# Autodesk Inventor assembly: Solarbotics-GM2_Assem
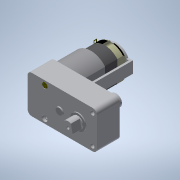
[picture p0: Inventor's stored thumbnail of the model, 180x180]
Saved by Autodesk Inventor 2020.1 (Build 241239000, 239)
## iProperties
Created: 2013-04-23
Part Number: Solarbotics-GM2_Assem
Document SubType Name: Assembly
Designer: justin
## Documents named in this file (7)
- C:\Users\amirs\OneDrive - UC San Diego\college\freshman year\MAE 3\robot\gm 2\Solarbotics-GM2_Assem.iam
- C:\Users\amirs\OneDrive - UC San Diego\college\freshman year\MAE 3\robot\gm 2\gm2.ipt
- C:\Users\amirs\OneDrive - UC San Diego\college\freshman year\MAE 3\robot\gm 2\RM3-regular motor.ipt
- C:\Users\amirs\OneDrive - UC San Diego\college\freshman year\MAE 3\robot\gm 2\GMstrap1.ipt
- C:\Users\amirs\OneDrive - UC San Diego\college\freshman year\MAE 3\robot\gm 2\screw_head1.ipt
- C:\Users\amirs\OneDrive - UC San Diego\college\freshman year\MAE 3\robot\gm 2\output shaft.ipt
- C:\Users\amirs\OneDrive - UC San Diego\college\freshman year\MAE 3\robot\gm 2\dshaft.ipt
## Components (6 placed, 6 different names)
1. gm2:1 — Flush:1, Flush:2, Flush:3, Insert:1, Insert:2
2. RM3-regular motor:1
3. GMstrap1:1 — Flush:1, Flush:2, Flush:3
4. screw_head1:1
5. output shaft:1 — Insert:1, Angle:1
6. dshaft:1 — Insert:2, Angle:1
## Relationships (6: Flush 3, Insert 2, Angle 1)
- Flush:1 (1.27 mm): gm2:1 ↔ GMstrap1:1
- Flush:2 (-7.615 mm): gm2:1 ↔ GMstrap1:1
- Flush:3 (-7.858 mm): gm2:1 ↔ GMstrap1:1
- Insert:1: gm2:1 ↔ output shaft:1
- Insert:2: gm2:1 ↔ dshaft:1
- Angle:1 (0 deg): output shaft:1 ↔ dshaft:1
